# Autodesk Inventor assembly: OBG_Dribbler
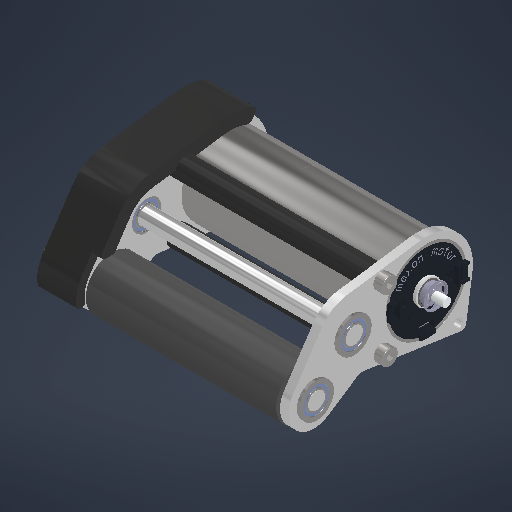
[picture p0: Inventor's stored thumbnail of the model, 512x512]
Saved by Autodesk Inventor 2025.2 (Build 292293000, 293)
## iProperties
Created: 2025-04-28
Part Number: OBG_Dribbler
Document SubType Name: Assembly
Designer: Faabs
Author: Faabs
## Documents named in this file (15)
- C:\Users\Faabs\Desktop\HBG v2023\OBG\Dribbler\OBG_Dribbler.iam
- C:\Users\Faabs\Desktop\HBG v2023\OBG\Dribbler\Dribblerseitenplatte_links\Dribblerseitenplatte_links\Dribblerseitenplatte_links.ipt
- C:\Users\Faabs\Desktop\HBG v2023\OBG\Dribbler\Dribblerseitenplatte_rechts\Dribblerseitenplatte_rechts\Dribblerseitenplatte_rechts.ipt
- C:\Users\Faabs\Desktop\HBG v2023\UBG\Antrieb\Maxon DCX 19mm 13W\DCX 19mm 13W.iam
- C:\Users\Faabs\Desktop\HBG v2023\OBG\Dribbler\Kugellager 4 x 7 x 2,5 mm\Kugellager 4 x 7 x 2,5 mm\Kugellager 4 x 7 x 2,5 mm.ipt
- C:\Users\Faabs\Desktop\HBG v2023\OBG\Dribbler\Dribblerwelle\Dribblerwelle\Dribblerwelle.ipt
- C:\Users\Faabs\Desktop\HBG v2023\OBG\Dribbler\Abstandshalter\Abstandshalter\Abstandshalter.ipt
- C:\Users\Faabs\Desktop\HBG v2023\OBG\Dribbler\Wellenaufsatz\Wellenaufsatz\Wellenaufsatz.ipt
- C:\Users\Faabs\Desktop\HBG v2023\OBG\Dribbler\Dribblergummi\Dribblergummi\Dribblergummi.ipt
- C:\Users\Faabs\Desktop\HBG v2023\Verbindungselemente\ISO 7046\DIN EN ISO 7046-2 H - M2x6 - 8.8 - H1.ipt
- C:\Users\Faabs\Desktop\HBG v2023\Verbindungselemente\DIN 912\DIN 912 - M2 x 0,4 x 6 x 5.ipt
- C:\Users\Faabs\Desktop\HBG v2023\OBG\Dribbler\Zahnradabdeckung\Zahnradabdeckung\Zahnradabdeckung.ipt
- C:\Users\Faabs\Desktop\HBG v2023\OBG\Dribbler\Zahnradabdeckung\Stirnzahnrad 20z\Stirnzahnrad 20z.ipt
- C:\Users\Faabs\Desktop\HBG v2023\OBG\Dribbler\Zahnradabdeckung\Stirnzahnrad 30z\Stirnzahnrad 30z.ipt
- C:\Users\Faabs\Desktop\HBG v2023\OBG\Dribbler\Zahnradabdeckung\Stirnzahnrad 40z\Stirnzahnrad 40z.ipt
## Components (24 placed, 14 different names)
1. DCX 19mm 13W:1 [sub-assembly] — Passend:1, Passend:2, Passend:3, Passend:4, Fluchtend:1, Fluchtend:2, Fluchtend:3, Passend:5, Fluchtend:4, Passend:27
2. Dribblerseitenplatte_links:1 — Passend:5, Passend:6, Fluchtend:4, Passend:7, Passend:8, Passend:9, Passend:10, Passend:17, Passend:18, Passend:19, Passend:20, Passend:22, Einfügen:4, Einfügen:5
3. Dribblerseitenplatte_rechts:1 — Passend:1, Passend:2, Passend:3, Passend:4, Passend:6, Passend:11, Passend:12, Passend:13, Passend:14, Einfügen:1, Einfügen:2, Einfügen:3, Passend:24, Passend:25, Passend:26, Einfügen:7
4. Kugellager 4 x 7 x 2,5 mm:1 — Passend:11, Passend:14
5. Kugellager 4 x 7 x 2,5 mm:2 — Passend:12, Passend:13, Passend:30
6. Kugellager 4 x 7 x 2,5 mm:3 — Passend:8, Passend:9, Passend:15
7. Kugellager 4 x 7 x 2,5 mm:4 — Passend:7, Passend:10, Passend:16
8. Dribblerwelle:1 — Passend:16, Fluchtend:5, Passend:21, Passend:29
9. Dribblerwelle:2 — Passend:15, Fluchtend:5, Passend:28
10. Abstandshalter:1 — Passend:17, Passend:19
11. Abstandshalter:2 — Passend:18, Passend:20
12. Wellenaufsatz:1 — Passend:21, Passend:22, Passend:23, Fluchtend:6
13. Dribblergummi:1 — Passend:23, Fluchtend:6
14. Zahnradabdeckung:1 — Passend:24, Passend:25, Passend:26, Einfügen:6
15. Stirnzahnrad 20z:1 — Passend:29, Fluchtend:7
16. Stirnzahnrad 30z:1 — Passend:28, Fluchtend:7, Fluchtend:8, Passend:30
17. Stirnzahnrad 40z:1 — Passend:27, Fluchtend:8
18. DIN EN ISO 7046-2 H M2x6 - 8.8 - H1:1 — Einfügen:3
19. DIN EN ISO 7046-2 H M2x6 - 8.8 - H1:2 — Einfügen:1
20. DIN EN ISO 7046-2 H M2x6 - 8.8 - H1:3 — Einfügen:2
21. DIN 912 - ersetzt durch DIN EN ISO 4762 M2 x 6:1 — Einfügen:4
22. DIN 912 - ersetzt durch DIN EN ISO 4762 M2 x 6:2 — Einfügen:5
23. DIN 912 - ersetzt durch DIN EN ISO 4762 M2 x 6:3 — Einfügen:7
24. DIN 912 - ersetzt durch DIN EN ISO 4762 M2 x 6:4 — Einfügen:6
## Relationships (45: Mate 30, Flush 8, Insert 7)
- Passend:1 [Mate]: DCX 19mm 13W:1 ↔ Dribblerseitenplatte_rechts:1
- Passend:2 [Mate]: DCX 19mm 13W:1 ↔ Dribblerseitenplatte_rechts:1
- Passend:3 [Mate]: DCX 19mm 13W:1 ↔ Dribblerseitenplatte_rechts:1
- Passend:4 [Mate]: DCX 19mm 13W:1 ↔ Dribblerseitenplatte_rechts:1
- Fluchtend:1 [Flush]: DCX 19mm 13W:1
- Fluchtend:2 [Flush]: DCX 19mm 13W:1
- Fluchtend:3 [Flush]: DCX 19mm 13W:1
- Passend:5 [Mate]: DCX 19mm 13W:1 ↔ Dribblerseitenplatte_links:1
- Passend:6 [Mate]: Dribblerseitenplatte_links:1 ↔ Dribblerseitenplatte_rechts:1
- Fluchtend:4 [Flush]: DCX 19mm 13W:1 ↔ Dribblerseitenplatte_links:1
- Passend:7 [Mate]: Dribblerseitenplatte_links:1 ↔ Kugellager 4 x 7 x 2,5 mm:4
- Passend:8 [Mate]: Dribblerseitenplatte_links:1 ↔ Kugellager 4 x 7 x 2,5 mm:3
- Passend:9 [Mate]: Dribblerseitenplatte_links:1 ↔ Kugellager 4 x 7 x 2,5 mm:3
- Passend:10 [Mate]: Dribblerseitenplatte_links:1 ↔ Kugellager 4 x 7 x 2,5 mm:4
- Passend:11 [Mate]: Dribblerseitenplatte_rechts:1 ↔ Kugellager 4 x 7 x 2,5 mm:1
- Passend:12 [Mate]: Dribblerseitenplatte_rechts:1 ↔ Kugellager 4 x 7 x 2,5 mm:2
- Passend:13 [Mate]: Dribblerseitenplatte_rechts:1 ↔ Kugellager 4 x 7 x 2,5 mm:2
- Passend:14 [Mate]: Dribblerseitenplatte_rechts:1 ↔ Kugellager 4 x 7 x 2,5 mm:1
- Passend:15 [Mate]: Kugellager 4 x 7 x 2,5 mm:3 ↔ Dribblerwelle:2
- Passend:16 [Mate]: Kugellager 4 x 7 x 2,5 mm:4 ↔ Dribblerwelle:1
- Fluchtend:5 [Flush]: Dribblerwelle:1 ↔ Dribblerwelle:2
- Passend:17 [Mate]: Dribblerseitenplatte_links:1 ↔ Abstandshalter:1
- Passend:18 [Mate]: Dribblerseitenplatte_links:1 ↔ Abstandshalter:2
- Passend:19 [Mate]: Dribblerseitenplatte_links:1 ↔ Abstandshalter:1
- Passend:20 [Mate]: Dribblerseitenplatte_links:1 ↔ Abstandshalter:2
- Passend:21 [Mate]: Dribblerwelle:1 ↔ Wellenaufsatz:1
- Passend:22 [Mate] (0.7 mm): Dribblerseitenplatte_links:1 ↔ Wellenaufsatz:1
- Passend:23 [Mate]: Wellenaufsatz:1 ↔ Dribblergummi:1
- Fluchtend:6 [Flush]: Wellenaufsatz:1 ↔ Dribblergummi:1
- Einfügen:1 [Insert]: Dribblerseitenplatte_rechts:1 ↔ DIN EN ISO 7046-2 H M2x6 - 8.8 - H1:2
- Einfügen:2 [Insert]: Dribblerseitenplatte_rechts:1 ↔ DIN EN ISO 7046-2 H M2x6 - 8.8 - H1:3
- Einfügen:3 [Insert]: Dribblerseitenplatte_rechts:1 ↔ DIN EN ISO 7046-2 H M2x6 - 8.8 - H1:1
- Einfügen:4 [Insert]: Dribblerseitenplatte_links:1 ↔ DIN 912 - ersetzt durch DIN EN ISO 4762 M2 x 6:1
- Einfügen:5 [Insert]: Dribblerseitenplatte_links:1 ↔ DIN 912 - ersetzt durch DIN EN ISO 4762 M2 x 6:2
- Passend:24 [Mate]: Dribblerseitenplatte_rechts:1 ↔ Zahnradabdeckung:1
- Passend:25 [Mate]: Dribblerseitenplatte_rechts:1 ↔ Zahnradabdeckung:1
- Passend:26 [Mate]: Dribblerseitenplatte_rechts:1 ↔ Zahnradabdeckung:1
- Einfügen:6 [Insert]: Zahnradabdeckung:1 ↔ DIN 912 - ersetzt durch DIN EN ISO 4762 M2 x 6:4
- Einfügen:7 [Insert]: Dribblerseitenplatte_rechts:1 ↔ DIN 912 - ersetzt durch DIN EN ISO 4762 M2 x 6:3
- Passend:27 [Mate]: DCX 19mm 13W:1 ↔ Stirnzahnrad 40z:1
- Passend:28 [Mate]: Dribblerwelle:2 ↔ Stirnzahnrad 30z:1
- Passend:29 [Mate]: Dribblerwelle:1 ↔ Stirnzahnrad 20z:1
- Fluchtend:7 [Flush]: Stirnzahnrad 20z:1 ↔ Stirnzahnrad 30z:1
- Fluchtend:8 [Flush]: Stirnzahnrad 30z:1 ↔ Stirnzahnrad 40z:1
- Passend:30 [Mate]: Kugellager 4 x 7 x 2,5 mm:2 ↔ Stirnzahnrad 30z:1
